# Autodesk Inventor assembly: Assembly5_turnsignal_back
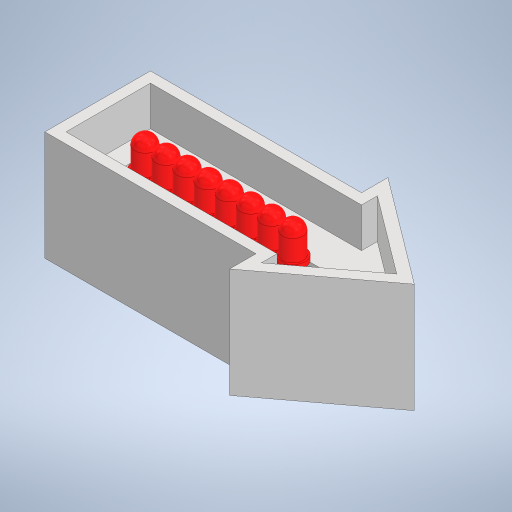
[picture p0: Inventor's stored thumbnail of the model, 512x512]
Saved by Autodesk Inventor 2023 (Build 270158000, 158)
## iProperties
Created: 2023-10-25
Part Number: Assembly5_turnsignal_back
Document SubType Name: Assembly
Designer: zskus
Author: zskus
## Documents named in this file (3)
- C:\Users\zskus\Desktop\Folders\Personal Projects\Inventor\Project_1_Scooter\Assembly\Assembly5_turnsignal_back.iam
- C:\Users\zskus\Desktop\Folders\Personal Projects\Inventor\Project_1_Scooter\Parts\Part_5_ledholder_back.ipt
- C:\Users\zskus\Desktop\Folders\Personal Projects\Inventor\Project_1_Scooter\Parts\red-led-5mm_MIR.ipt
## Components (9 placed, 2 different names)
1. Part_5_ledholder_back:1 — Mate:1, Mate:2
2. red-led-5mm_MIR:1 — Mate:1, Mate:2
3. red-led-5mm_MIR:2
4. red-led-5mm_MIR:3
5. red-led-5mm_MIR:4
6. red-led-5mm_MIR:5
7. red-led-5mm_MIR:6
8. red-led-5mm_MIR:7
9. red-led-5mm_MIR:8
## Component patterns: (8 elements, first: red-led-5mm_MIR:1)
## Relationships (2: Mate 2)
- Mate:1: Part_5_ledholder_back:1 ↔ red-led-5mm_MIR:1
- Mate:2: Part_5_ledholder_back:1 ↔ red-led-5mm_MIR:1
